# Autodesk Inventor assembly: Manual_Robot
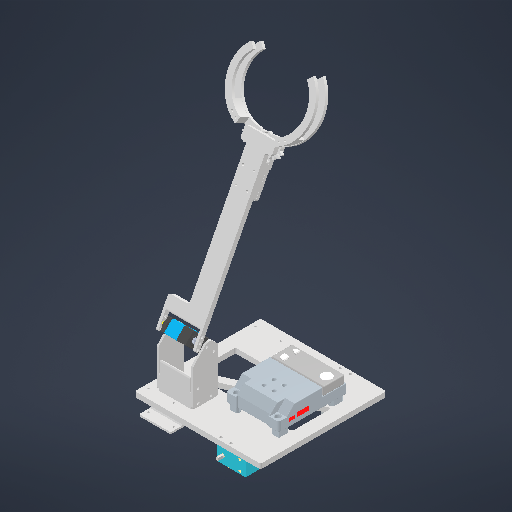
[picture p0: Inventor's stored thumbnail of the model, 512x512]
Saved by Autodesk Inventor 2026.1 (Build 301233020, 233B)
## iProperties
Created: 2025-10-29
Part Number: Manual_Robot
Document SubType Name: Assembly
Designer: Garfieldcmix
Author: Garfieldcmix
## Documents named in this file (9)
- C:\Users\Garfieldcmix\git\KMITL-ComPro-Group-Work\models\manual-robot\Manual_Robot.iam
- C:\Users\Garfieldcmix\git\KMITL-ComPro-Group-Work\models\manual-robot\Chassis.ipt
- C:\Users\Garfieldcmix\git\KMITL-ComPro-Group-Work\models\manual-robot\components\mbot2_shield.ipt
- C:\Users\Garfieldcmix\git\KMITL-ComPro-Group-Work\models\manual-robot\components\cyberpi.ipt
- C:\Users\Garfieldcmix\git\KMITL-ComPro-Group-Work\models\manual-robot\components\encoder_motor.ipt
- C:\Users\Garfieldcmix\git\KMITL-ComPro-Group-Work\models\manual-robot\Arm_Servo_Holder.ipt
- C:\Users\Garfieldcmix\git\KMITL-ComPro-Group-Work\models\manual-robot\components\MEDS15_Servo_Motor.ipt
- C:\Users\Garfieldcmix\git\KMITL-ComPro-Group-Work\models\manual-robot\Arm_Assembly.iam
- C:\Users\Garfieldcmix\git\KMITL-ComPro-Group-Work\models\manual-robot\Front_Wheel_Stand.ipt
## Components (11 placed, 8 different names)
1. Chassis:1 — Mate:1, Mate:2, Mate:3, Mate:7, Mate:8, Mate:9, Mate:10, Mate:11, Mate:12, Mate:13, Mate:14, Mate:15, Mate:16, Mate:17, Mate:18, Mate:22, Mate:23, Mate:24, Mate:25, Mate:26, Mate:27
2. mbot2_shield:1 — Mate:1, Mate:2, Mate:3, Mate:4, Mate:5, Mate:6
3. cyberpi:1 — Mate:4, Mate:5, Mate:6
4. encoder_motor:1 — Mate:7, Mate:8, Mate:9
5. encoder_motor:2 — Mate:10, Mate:11, Mate:12
6. Arm_Servo_Holder:1 — Mate:13, Mate:14, Mate:15, Mate:19, Mate:20, Mate:21, Flush:1
7. Arm_Servo_Holder:2 — Mate:16, Mate:17, Mate:18
8. MEDS15_Servo_Motor:1 — Mate:19, Mate:20, Mate:21, Cylindrical:1
9. Arm_Assembly:1 [sub-assembly] — Cylindrical:1, Flush:1
10. Front_Wheel_Stand:1 — Mate:22, Mate:23, Mate:24
11. Front_Wheel_Stand:2 — Mate:25, Mate:26, Mate:27
## Relationships (29: Mate 27, CylindricalJoint 1, Flush 1)
- Mate:1: Chassis:1 ↔ mbot2_shield:1
- Mate:2: Chassis:1 ↔ mbot2_shield:1
- Mate:3: Chassis:1 ↔ mbot2_shield:1
- Mate:4: mbot2_shield:1 ↔ cyberpi:1
- Mate:5: mbot2_shield:1 ↔ cyberpi:1
- Mate:6: mbot2_shield:1 ↔ cyberpi:1
- Mate:7: Chassis:1 ↔ encoder_motor:1
- Mate:8: Chassis:1 ↔ encoder_motor:1
- Mate:9: Chassis:1 ↔ encoder_motor:1
- Mate:10: Chassis:1 ↔ encoder_motor:2
- Mate:11: Chassis:1 ↔ encoder_motor:2
- Mate:12: Chassis:1 ↔ encoder_motor:2
- Mate:13: Chassis:1 ↔ Arm_Servo_Holder:1
- Mate:14: Chassis:1 ↔ Arm_Servo_Holder:1
- Mate:15: Chassis:1 ↔ Arm_Servo_Holder:1
- Mate:16: Chassis:1 ↔ Arm_Servo_Holder:2
- Mate:17: Chassis:1 ↔ Arm_Servo_Holder:2
- Mate:18: Chassis:1 ↔ Arm_Servo_Holder:2
- Mate:19: Arm_Servo_Holder:1 ↔ MEDS15_Servo_Motor:1
- Mate:20: Arm_Servo_Holder:1 ↔ MEDS15_Servo_Motor:1
- Mate:21: Arm_Servo_Holder:1 ↔ MEDS15_Servo_Motor:1
- Cylindrical:1: MEDS15_Servo_Motor:1 ↔ Arm_Assembly:1
- Flush:1: Arm_Servo_Holder:1 ↔ Arm_Assembly:1
- Mate:22: Chassis:1 ↔ Front_Wheel_Stand:1
- Mate:23: Chassis:1 ↔ Front_Wheel_Stand:1
- Mate:24: Chassis:1 ↔ Front_Wheel_Stand:1
- Mate:25: Chassis:1 ↔ Front_Wheel_Stand:2
- Mate:26: Chassis:1 ↔ Front_Wheel_Stand:2
- Mate:27: Chassis:1 ↔ Front_Wheel_Stand:2
